# Autodesk Inventor assembly: FullMotor
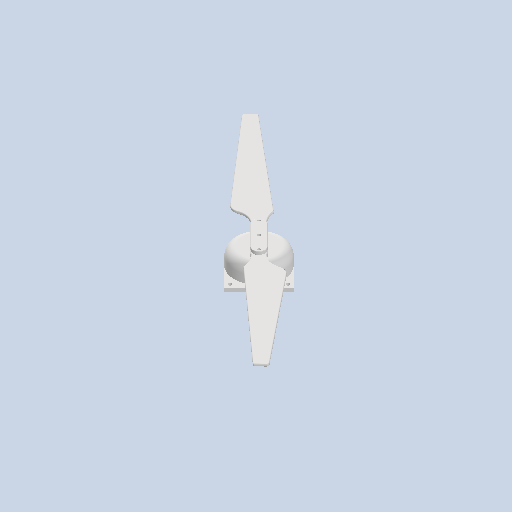
[picture p0: Inventor's stored thumbnail of the model, 512x512]
Saved by Autodesk Inventor 2022.1 (Build 261234020, 234B)
## iProperties
Created: 2022-10-16
Part Number: FullMotor
Document SubType Name: Assembly
Designer: Alexander
Author: Alexander
## Documents named in this file (4)
- C:\Users\Alexander\Desktop\Drone\inventor\Propeller\FullMotor.iam
- C:\Users\Alexander\Desktop\Drone\inventor\Propeller\Motor.ipt
- C:\Users\Alexander\Desktop\Drone\inventor\Propeller\FullProp.iam
- C:\Users\Alexander\Desktop\Drone\inventor\Propeller\MotorBasePlate.ipt
## Components (3 placed, 3 different names)
1. Motor:1 — Rotational:1, Mate:1, Mate:2, Mate:3
2. FullProp:1 [sub-assembly] — Rotational:1
3. MotorBasePlate:1 — Mate:1, Mate:2, Mate:3
## Relationships (4: Mate 3, RevoluteJoint 1)
- Rotational:1 [RevoluteJoint]: Motor:1 ↔ FullProp:1
- Mate:1: Motor:1 ↔ MotorBasePlate:1
- Mate:2: Motor:1 ↔ MotorBasePlate:1
- Mate:3: Motor:1 ↔ MotorBasePlate:1
